# Autodesk Inventor assembly: cabeça_inferior
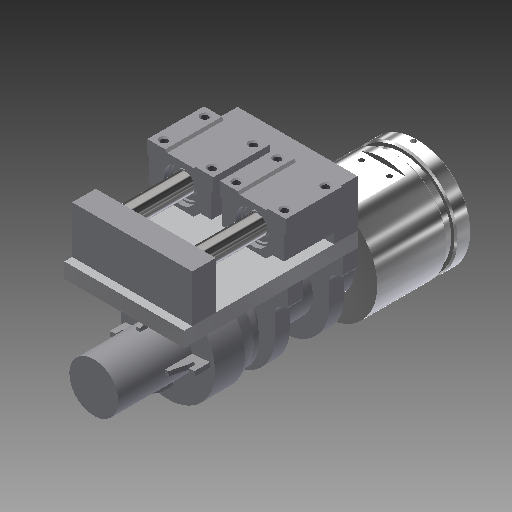
[picture p0: Inventor's stored thumbnail of the model, 512x512]
Saved by Autodesk Inventor 2018 (Build 220112000, 112)
## iProperties
Created: 2018-05-10
Part Number: cabeça_inferior
Material: Genérico
Document SubType Name: Assembly
Designer: Georgines
Mass: 1069.3 g
Surface Area: 1697.31 cm^2
Volume: 551.873 cm^3
Density: 1.93759 g/cm^3
Author: Georgines
## Documents named in this file (8)
- C:\Users\Usuario\Desktop\pecas_3d-20180530T120808Z-001\pecas_3d\cabeça_inferior.iam
- C:\Users\Usuario\Desktop\pecas_3d-20180530T120808Z-001\pecas_3d\bocal_de_aquecimento.ipt
- C:\Users\Usuario\Desktop\pecas_3d-20180530T120808Z-001\pecas_3d\soprador_original.ipt
- C:\Users\Usuario\Desktop\pecas_3d-20180530T120808Z-001\pecas_3d\suporte_boca_soprador.ipt
- C:\Users\Usuario\Desktop\pecas_3d-20180530T120808Z-001\pecas_3d\SCS12UU.iam
- C:\Users\Usuario\Desktop\pecas_3d-20180530T120808Z-001\pecas_3d\SuporteAquecedor.ipt
- C:\Users\Usuario\Desktop\pecas_3d-20180530T120808Z-001\pecas_3d\guia_linear_12mm_150mm.ipt
- C:\Users\Usuario\Desktop\pecas_3d-20180530T120808Z-001\pecas_3d\SuporteGuiasCabeçasAquecimento.ipt
## Components (11 placed, 7 different names)
1. bocal_de_aquecimento:1 — Inserir:1, Alinhamento:2
2. soprador_original:1 — Inserir:1, Coincidência:3
3. suporte_boca_soprador:1 — Alinhamento:2, Coincidência:1, Coincidência:2, Alinhamento:3, Alinhamento:4, Alinhamento:5, Coincidência:12, Alinhamento:9, Alinhamento:10
4. SCS12UU:1 [sub-assembly] — Coincidência:10, Alinhamento:7, Alinhamento:8
5. SCS12UU:2 [sub-assembly] — Coincidência:11, Alinhamento:7, Alinhamento:8
6. SuporteAquecedor:1 — Coincidência:2, Alinhamento:3
7. SuporteAquecedor:2 — Coincidência:1, Alinhamento:4, Coincidência:3, Alinhamento:5
8. guia_linear_12mm_150mm:1 — Coincidência:5, Alinhamento:6, Coincidência:8, Coincidência:11
9. guia_linear_12mm_150mm:2 — Coincidência:4, Alinhamento:6, Coincidência:6, Coincidência:7, Coincidência:9, Coincidência:10
10. SuporteGuiasCabeçasAquecimento:1 — Coincidência:7, Coincidência:8, Coincidência:9, Coincidência:12, Alinhamento:9, Alinhamento:10
11. SuporteGuiasCabeçasAquecimento:2 — Coincidência:4, Coincidência:5, Coincidência:6
## Relationships (22: Mate 12, Flush 9, Insert 1)
- Inserir:1 (-2.5 mm): bocal_de_aquecimento:1 ↔ soprador_original:1
- Alinhamento:2 [Flush]: bocal_de_aquecimento:1 ↔ suporte_boca_soprador:1
- Coincidência:1 [Mate]: suporte_boca_soprador:1 ↔ SuporteAquecedor:2
- Coincidência:2 [Mate]: suporte_boca_soprador:1 ↔ SuporteAquecedor:1
- Alinhamento:3 [Flush]: suporte_boca_soprador:1 ↔ SuporteAquecedor:1
- Alinhamento:4 [Flush]: suporte_boca_soprador:1 ↔ SuporteAquecedor:2
- Coincidência:3 [Mate]: soprador_original:1 ↔ SuporteAquecedor:2
- Alinhamento:5 [Flush]: suporte_boca_soprador:1 ↔ SuporteAquecedor:2
- Coincidência:4 [Mate]: guia_linear_12mm_150mm:2 ↔ SuporteGuiasCabeçasAquecimento:2
- Coincidência:5 [Mate]: guia_linear_12mm_150mm:1 ↔ SuporteGuiasCabeçasAquecimento:2
- Alinhamento:6 [Flush]: guia_linear_12mm_150mm:1 ↔ guia_linear_12mm_150mm:2
- Coincidência:6 [Mate]: guia_linear_12mm_150mm:2 ↔ SuporteGuiasCabeçasAquecimento:2
- Coincidência:7 [Mate]: guia_linear_12mm_150mm:2 ↔ SuporteGuiasCabeçasAquecimento:1
- Coincidência:8 [Mate]: guia_linear_12mm_150mm:1 ↔ SuporteGuiasCabeçasAquecimento:1
- Coincidência:9 [Mate]: guia_linear_12mm_150mm:2 ↔ SuporteGuiasCabeçasAquecimento:1
- Coincidência:10 [Mate]: SCS12UU:1 ↔ guia_linear_12mm_150mm:2
- Coincidência:11 [Mate]: SCS12UU:2 ↔ guia_linear_12mm_150mm:1
- Alinhamento:7 [Flush]: SCS12UU:1 ↔ SCS12UU:2
- Alinhamento:8 [Flush]: SCS12UU:1 ↔ SCS12UU:2
- Coincidência:12 [Mate]: suporte_boca_soprador:1 ↔ SuporteGuiasCabeçasAquecimento:1
- Alinhamento:9 [Flush]: suporte_boca_soprador:1 ↔ SuporteGuiasCabeçasAquecimento:1
- Alinhamento:10 [Flush] (5 mm): suporte_boca_soprador:1 ↔ SuporteGuiasCabeçasAquecimento:1
